# Autodesk Inventor assembly: main_assembly
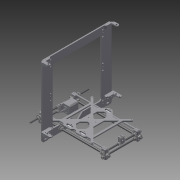
[picture p0: Inventor's stored thumbnail of the model, 180x180]
Saved by Autodesk Inventor 2015 (Build 190159000, 159)
## iProperties
Created: 2015-05-09
Part Number: main_assembly
Document SubType Name: Assembly
Designer: X
Author: X
## Documents named in this file (9)
- G:\3d printer\Prusa_i3\CAD\main_assembly.iam
- G:\3d printer\Prusa_i3\CAD\frame\platform_redrawn.ipt
- G:\3d printer\Prusa_i3\CAD\3d_printer_part\y-belt-holder.ipt
- G:\3d printer\Prusa_i3\CAD\chassis.iam
- G:\3d printer\Prusa_i3\CAD\standard_parts\Imported Components\NEMA 17 Stepper Motor Assembly\NEMA 17 Stepper Motor Assembly.iam
- G:\3d printer\Prusa_i3\CAD\standard_parts\LM8UU 8mm Linear Bearing.ipt
- G:\3d printer\Prusa_i3\CAD\main_frame_assem.iam
- D:\Inventor\Content Center Files\R2015\en-US\ISO 7093 A\ISO 7093 A - ST 10 - 140 HV .ipt
- D:\Inventor\Content Center Files\R2015\en-US\DIN 934\DIN 934 - M10 x 1.5.ipt
## Components (16 placed, 8 different names)
1. platform_redrawn:1 — Cylindrical:1, Cylindrical:2, Mate:1, Angle:1, Mate:3, Tangent:1, Tangent:2, Mate:4, Mate:5
2. y-belt-holder:1 — Cylindrical:1, Cylindrical:2, Mate:1
3. chassis:1 [sub-assembly] — Cylindrical:3, Cylindrical:4, Mate:2, Cylindrical:5, Cylindrical:6, Cylindrical:7, Angle:1, Mate:6, Mate:7, Cylindrical:8, Cylindrical:9, Cylindrical:10, Cylindrical:11, Cylindrical:12, Cylindrical:13, Cylindrical:14, Cylindrical:15, Cylindrical:16, Cylindrical:17
4. NEMA 17 Stepper Motor Assembly:1 [sub-assembly] — Cylindrical:3, Cylindrical:4, Mate:2
5. LM8UU 8mm Linear Bearing:1 — Cylindrical:6, Mate:3, Tangent:1, Tangent:2
6. LM8UU 8mm Linear Bearing:2 — Cylindrical:5, Mate:4
7. LM8UU 8mm Linear Bearing:3 — Cylindrical:7, Mate:5
8. main_frame_assem:1 [sub-assembly] — Cylindrical:8, Cylindrical:9, Mate:8, Mate:9, Mate:10, Mate:11
9. ISO 7093 A ST 10 - 140 HV - A:1 — Cylindrical:12, Mate:9, Mate:12
10. ISO 7093 A ST 10 - 140 HV - A:2 — Cylindrical:13, Mate:10, Mate:13
11. ISO 7093 A ST 10 - 140 HV - A:3 — Cylindrical:10, Mate:8, Mate:15
12. ISO 7093 A ST 10 - 140 HV - A:4 — Cylindrical:11, Mate:11, Mate:14
13. DIN 934 - replaced by DIN EN 24032/28673/28674 M10:1 — Cylindrical:14, Mate:12
14. DIN 934 - replaced by DIN EN 24032/28673/28674 M10:2 — Cylindrical:15, Mate:13
15. DIN 934 - replaced by DIN EN 24032/28673/28674 M10:3 — Cylindrical:17, Mate:15
16. DIN 934 - replaced by DIN EN 24032/28673/28674 M10:4 — Cylindrical:16, Mate:14
## Relationships (35: CylindricalJoint 17, Mate 15, Tangent 2, Angle 1)
- Cylindrical:1: platform_redrawn:1 ↔ y-belt-holder:1
- Cylindrical:2: platform_redrawn:1 ↔ y-belt-holder:1
- Mate:1: platform_redrawn:1 ↔ y-belt-holder:1
- Cylindrical:3: chassis:1 ↔ NEMA 17 Stepper Motor Assembly:1
- Cylindrical:4: chassis:1 ↔ NEMA 17 Stepper Motor Assembly:1
- Mate:2: chassis:1 ↔ NEMA 17 Stepper Motor Assembly:1
- Cylindrical:5: chassis:1 ↔ LM8UU 8mm Linear Bearing:2
- Cylindrical:6: chassis:1 ↔ LM8UU 8mm Linear Bearing:1
- Cylindrical:7: chassis:1 ↔ LM8UU 8mm Linear Bearing:3
- Angle:1 (0 deg): platform_redrawn:1 ↔ chassis:1
- Mate:3 (3.5 mm): platform_redrawn:1 ↔ LM8UU 8mm Linear Bearing:1
- Tangent:1: platform_redrawn:1 ↔ LM8UU 8mm Linear Bearing:1
- Tangent:2: platform_redrawn:1 ↔ LM8UU 8mm Linear Bearing:1
- Mate:4 (3.5 mm): platform_redrawn:1 ↔ LM8UU 8mm Linear Bearing:2
- Mate:5 (3.5 mm): platform_redrawn:1 ↔ LM8UU 8mm Linear Bearing:3
- Mate:6: chassis:1
- Mate:7: chassis:1
- Cylindrical:8: chassis:1 ↔ main_frame_assem:1
- Cylindrical:9: chassis:1 ↔ main_frame_assem:1
- Cylindrical:10: chassis:1 ↔ ISO 7093 A ST 10 - 140 HV - A:3
- Cylindrical:11: chassis:1 ↔ ISO 7093 A ST 10 - 140 HV - A:4
- Cylindrical:12: chassis:1 ↔ ISO 7093 A ST 10 - 140 HV - A:1
- Cylindrical:13: chassis:1 ↔ ISO 7093 A ST 10 - 140 HV - A:2
- Mate:8: main_frame_assem:1 ↔ ISO 7093 A ST 10 - 140 HV - A:3
- Mate:9: main_frame_assem:1 ↔ ISO 7093 A ST 10 - 140 HV - A:1
- Mate:10: main_frame_assem:1 ↔ ISO 7093 A ST 10 - 140 HV - A:2
- Mate:11: main_frame_assem:1 ↔ ISO 7093 A ST 10 - 140 HV - A:4
- Cylindrical:14: chassis:1 ↔ DIN 934 - replaced by DIN EN 24032/28673/28674 M10:1
- Cylindrical:15: chassis:1 ↔ DIN 934 - replaced by DIN EN 24032/28673/28674 M10:2
- Cylindrical:16: chassis:1 ↔ DIN 934 - replaced by DIN EN 24032/28673/28674 M10:4
- Cylindrical:17: chassis:1 ↔ DIN 934 - replaced by DIN EN 24032/28673/28674 M10:3
- Mate:12: ISO 7093 A ST 10 - 140 HV - A:1 ↔ DIN 934 - replaced by DIN EN 24032/28673/28674 M10:1
- Mate:13: ISO 7093 A ST 10 - 140 HV - A:2 ↔ DIN 934 - replaced by DIN EN 24032/28673/28674 M10:2
- Mate:14: ISO 7093 A ST 10 - 140 HV - A:4 ↔ DIN 934 - replaced by DIN EN 24032/28673/28674 M10:4
- Mate:15: ISO 7093 A ST 10 - 140 HV - A:3 ↔ DIN 934 - replaced by DIN EN 24032/28673/28674 M10:3
